# Autodesk Inventor assembly: Base 03
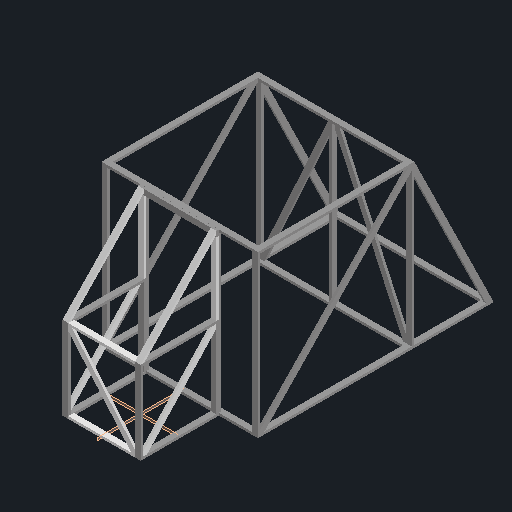
[picture p0: Inventor's stored thumbnail of the model, 512x512]
Saved by Autodesk Inventor 2026 (Build 300175000, 175)
## iProperties
Created: 2024-09-19
Part Number: Base 03
Document SubType Name: Assembly
Designer: User
Author: User
## Documents named in this file (13)
- C:\Users\trott\Documents\UofSC-ASME-Tiger-Burn-Design-2025\CAD\Body\Base 03\Base 03.iam
- C:\Users\trott\Documents\UofSC-ASME-Tiger-Burn-Design-2025\CAD\Body\Base 03\2x4x144.ipt
- C:\Users\trott\Documents\UofSC-ASME-Tiger-Burn-Design-2025\CAD\Body\Base 03\2x4x90.ipt
- C:\Users\trott\Documents\UofSC-ASME-Tiger-Burn-Design-2025\CAD\Body\Base 03\2x4x96.ipt
- C:\Users\trott\Documents\UofSC-ASME-Tiger-Burn-Design-2025\CAD\Body\Base 03\S_2x4x48b.ipt
- C:\Users\trott\Documents\UofSC-ASME-Tiger-Burn-Design-2025\CAD\Body\Base 03\S_2x4x88.ipt
- C:\Users\trott\Documents\UofSC-ASME-Tiger-Burn-Design-2025\CAD\Body\Base 03\S_2x4x48a.ipt
- C:\Users\trott\Documents\UofSC-ASME-Tiger-Burn-Design-2025\CAD\Reference (TB24)\F_Legs2\4x2x4.ipt
- C:\Users\trott\Documents\UofSC-ASME-Tiger-Burn-Design-2025\CAD\Body\Base 03\2x4x41.ipt
- C:\Users\trott\Documents\UofSC-ASME-Tiger-Burn-Design-2025\CAD\Body\Base 03\2x4x44.5.ipt
- C:\Users\trott\Documents\UofSC-ASME-Tiger-Burn-Design-2025\CAD\Body\Base 03\S_2x4x66.83.ipt
- C:\Users\trott\Documents\UofSC-ASME-Tiger-Burn-Design-2025\CAD\Body\Base 03\S_2x4x65.795.ipt
- C:\Users\trott\Documents\UofSC-ASME-Tiger-Burn-Design-2025\CAD\Body\Base 03\S_2x4x63.127.ipt
## Components (40 placed, 12 different names)
1. 2x4x144:1 — Flush:3, Flush:4, Flush:5, Mate:2, Mate:3, Mate:5, Flush:15, Flush:16, Flush:17, Flush:38, Flush:41
2. 2x4x144:2 — Flush:3, Flush:4, Flush:5, Mate:1, Flush:6, Flush:7, Flush:8, Flush:9, Flush:10, Mate:4, Mate:6, Flush:12, Flush:13, Flush:14, Mate:24, Flush:43
3. 2x4x90:1 — Mate:1, Flush:6, Flush:7, Flush:11, Mate:25, Flush:40, Mate:26, Flush:42
4. 2x4x90:2 — Flush:10, Flush:11, Flush:18, Flush:19, Mate:11, Flush:28
5. 2x4x90:3 — Flush:8, Flush:9, Mate:2
6. 2x4x96:1 — Mate:4, Flush:13, Flush:14, Mate:8, Flush:21, Flush:22, Flush:36
7. 2x4x96:2 — Mate:3, Flush:15, Flush:16, Mate:7, Flush:20, Flush:23
8. 2x4x96:3 — Mate:5, Flush:17, Flush:18, Flush:31, Mate:22
9. 2x4x96:4 — Mate:6, Flush:12, Flush:19, Mate:23, Flush:39
10. 2x4x96:5 — Mate:8, Flush:21, Flush:22, Mate:9, Flush:26, Mate:10, Flush:27
11. 2x4x96:6 — Mate:7, Flush:20, Flush:23, Flush:24, Flush:25, Mate:21, Flush:37
12. 2x4x90:4 — Flush:24, Mate:10, Flush:27, Mate:35, Flush:63, Mate:44
13. 2x4x90:5 — Flush:25, Mate:9, Flush:26, Mate:18, Mate:20
14. 2x4x96:8 — Mate:11, Flush:28, Flush:31, Mate:17, Flush:34, Mate:19, Flush:35
15. S_2x4x48b:3 — Mate:17, Mate:18, Flush:34
16. S_2x4x48b:4 — Mate:19, Mate:20, Flush:35
17. S_2x4x88:1 — Flush:36
18. S_2x4x88:2 — Mate:21, Mate:22, Flush:37
19. S_2x4x48a:1 — Flush:38
20. S_2x4x48a:2 — Mate:23, Mate:24, Flush:39
21. 4x2x4:1 — Mate:25, Flush:40, Flush:41, Flush:44, Flush:46, Mate:28, Flush:47, Flush:48
22. 4x2x4:2 — Mate:26, Flush:42, Flush:43, Mate:27, Flush:45, Flush:49
23. 2x4x41:1 — Flush:44, Mate:27, Flush:45, Flush:56
24. 4x2x4:3 — Flush:46, Mate:28, Flush:47, Flush:48, Flush:52, Mate:30, Flush:53, Flush:66, Mate:38
25. 4x2x4:4 — Flush:54, Mate:31, Flush:55, Mate:32, Flush:57, Mate:42, Mate:43, Flush:71, Flush:72
26. 4x2x4:5 — Flush:52, Mate:30, Flush:53, Mate:41
27. 2x4x41:2 — Flush:54, Mate:31, Flush:55
28. 2x4x44.5:1 — Mate:32, Flush:57, Flush:59, Mate:33, Flush:60, Flush:61, Flush:62
29. 4x2x4:6 — Flush:59, Mate:33, Flush:60, Mate:34, Mate:40, Mate:45
30. S_2x4x66.83:1 — Mate:34, Flush:61
31. 2x4x96:1 — Mate:35, Flush:62, Flush:63, Flush:70
32. S_2x4x65.795:1
33. S_2x4x65.795:2
34. S_2x4x63.127:1 — Flush:66, Mate:38
35. 2x4x44.5:2 — Mate:40, Flush:74
36. 4x2x4:7 — Mate:41, Flush:73
37. 4x2x4:8 — Mate:42, Flush:70
38. 4x2x4:9 — Mate:43, Flush:71, Flush:72
39. 2x4x96:10 — Mate:44, Flush:73
40. S_2x4x66.83:2 — Mate:45, Flush:74
## Relationships (96: Flush 60, Mate 36)
- Flush:3 (2349.5 mm): 2x4x144:1 ↔ 2x4x144:2
- Flush:4: 2x4x144:1 ↔ 2x4x144:2
- Flush:5: 2x4x144:1 ↔ 2x4x144:2
- Mate:1: 2x4x144:2 ↔ 2x4x90:1
- Flush:6: 2x4x144:2 ↔ 2x4x90:1
- Flush:7: 2x4x144:2 ↔ 2x4x90:1
- Flush:8: 2x4x144:2 ↔ 2x4x90:3
- Flush:9: 2x4x144:2 ↔ 2x4x90:3
- Mate:2: 2x4x144:1 ↔ 2x4x90:3
- Flush:10: 2x4x144:2 ↔ 2x4x90:2
- Flush:11 (2349.5 mm): 2x4x90:1 ↔ 2x4x90:2
- Mate:3: 2x4x144:1 ↔ 2x4x96:2
- Mate:4: 2x4x144:2 ↔ 2x4x96:1
- Mate:5: 2x4x144:1 ↔ 2x4x96:3
- Mate:6: 2x4x144:2 ↔ 2x4x96:4
- Flush:12: 2x4x144:2 ↔ 2x4x96:4
- Flush:13: 2x4x144:2 ↔ 2x4x96:1
- Flush:14: 2x4x144:2 ↔ 2x4x96:1
- Flush:15: 2x4x144:1 ↔ 2x4x96:2
- Flush:16: 2x4x144:1 ↔ 2x4x96:2
- Flush:17: 2x4x144:1 ↔ 2x4x96:3
- Flush:18: 2x4x90:2 ↔ 2x4x96:3
- Flush:19: 2x4x90:2 ↔ 2x4x96:4
- Mate:7: 2x4x96:2 ↔ 2x4x96:6
- Mate:8: 2x4x96:1 ↔ 2x4x96:5
- Flush:20: 2x4x96:2 ↔ 2x4x96:6
- Flush:21: 2x4x96:1 ↔ 2x4x96:5
- Flush:22: 2x4x96:1 ↔ 2x4x96:5
- Flush:23: 2x4x96:2 ↔ 2x4x96:6
- Flush:24: 2x4x96:6 ↔ 2x4x90:4
- Flush:25: 2x4x96:6 ↔ 2x4x90:5
- Mate:9: 2x4x96:5 ↔ 2x4x90:5
- Flush:26: 2x4x96:5 ↔ 2x4x90:5
- Mate:10: 2x4x96:5 ↔ 2x4x90:4
- Flush:27: 2x4x96:5 ↔ 2x4x90:4
- Mate:11: 2x4x90:2 ↔ 2x4x96:8
- Flush:28: 2x4x90:2 ↔ 2x4x96:8
- Flush:31 (1200.15 mm): 2x4x96:3 ↔ 2x4x96:8
- Mate:17: 2x4x96:8 ↔ S_2x4x48b:3
- Mate:18: 2x4x90:5 ↔ S_2x4x48b:3
- Flush:34: 2x4x96:8 ↔ S_2x4x48b:3
- Mate:19: 2x4x96:8 ↔ S_2x4x48b:4
- Mate:20: 2x4x90:5 ↔ S_2x4x48b:4
- Flush:35: 2x4x96:8 ↔ S_2x4x48b:4
- Flush:36: 2x4x96:1 ↔ S_2x4x88:1
- Mate:21: 2x4x96:6 ↔ S_2x4x88:2
- Mate:22: 2x4x96:3 ↔ S_2x4x88:2
- Flush:37: 2x4x96:6 ↔ S_2x4x88:2
- Flush:38: 2x4x144:1 ↔ S_2x4x48a:1
- Mate:23: 2x4x96:4 ↔ S_2x4x48a:2
- Mate:24: 2x4x144:2 ↔ S_2x4x48a:2
- Flush:39: 2x4x96:4 ↔ S_2x4x48a:2
- Mate:25: 2x4x90:1 ↔ 4x2x4:1
- Flush:40: 2x4x90:1 ↔ 4x2x4:1
- Flush:41 (609.6 mm): 2x4x144:1 ↔ 4x2x4:1
- Mate:26: 2x4x90:1 ↔ 4x2x4:2
- Flush:42: 2x4x90:1 ↔ 4x2x4:2
- Flush:43 (609.6 mm): 2x4x144:2 ↔ 4x2x4:2
- Flush:44: 4x2x4:1 ↔ 2x4x41:1
- Mate:27: 4x2x4:2 ↔ 2x4x41:1
- Flush:45: 4x2x4:2 ↔ 2x4x41:1
- Flush:46: 4x2x4:1 ↔ 4x2x4:3
- Mate:28: 4x2x4:1 ↔ 4x2x4:3
- Flush:47: 4x2x4:1 ↔ 4x2x4:3
- Flush:48: 4x2x4:1 ↔ 4x2x4:3
- Flush:49 (-609.6 mm): 4x2x4:2
- Flush:52: 4x2x4:3 ↔ 4x2x4:5
- Mate:30: 4x2x4:3 ↔ 4x2x4:5
- Flush:53: 4x2x4:3 ↔ 4x2x4:5
- Flush:54: 4x2x4:4 ↔ 2x4x41:2
- Mate:31: 4x2x4:4 ↔ 2x4x41:2
- Flush:55: 4x2x4:4 ↔ 2x4x41:2
- Flush:56 (-609.6 mm): 2x4x41:1
- Mate:32: 4x2x4:4 ↔ 2x4x44.5:1
- Flush:57: 4x2x4:4 ↔ 2x4x44.5:1
- Flush:59: 2x4x44.5:1 ↔ 4x2x4:6
- Mate:33: 2x4x44.5:1 ↔ 4x2x4:6
- Flush:60: 2x4x44.5:1 ↔ 4x2x4:6
- Mate:34: 4x2x4:6 ↔ S_2x4x66.83:1
- Flush:61: 2x4x44.5:1 ↔ S_2x4x66.83:1
- Mate:35: 2x4x90:4 ↔ 2x4x96:1
- Flush:62: 2x4x44.5:1 ↔ 2x4x96:1
- Flush:63: 2x4x90:4 ↔ 2x4x96:1
- Flush:66: 4x2x4:3 ↔ S_2x4x63.127:1
- Mate:38: 4x2x4:3 ↔ S_2x4x63.127:1
- Mate:40: 4x2x4:6 ↔ 2x4x44.5:2
- Mate:41: 4x2x4:5 ↔ 4x2x4:7
- Mate:42: 4x2x4:4 ↔ 4x2x4:8
- Flush:70: 2x4x96:1 ↔ 4x2x4:8
- Mate:43: 4x2x4:4 ↔ 4x2x4:9
- Flush:71: 4x2x4:4 ↔ 4x2x4:9
- Flush:72: 4x2x4:4 ↔ 4x2x4:9
- Mate:44: 2x4x90:4 ↔ 2x4x96:10
- Flush:73: 4x2x4:7 ↔ 2x4x96:10
- Mate:45: 4x2x4:6 ↔ S_2x4x66.83:2
- Flush:74: 2x4x44.5:2 ↔ S_2x4x66.83:2
